# Autodesk Inventor assembly: base mg996r 3mm with top
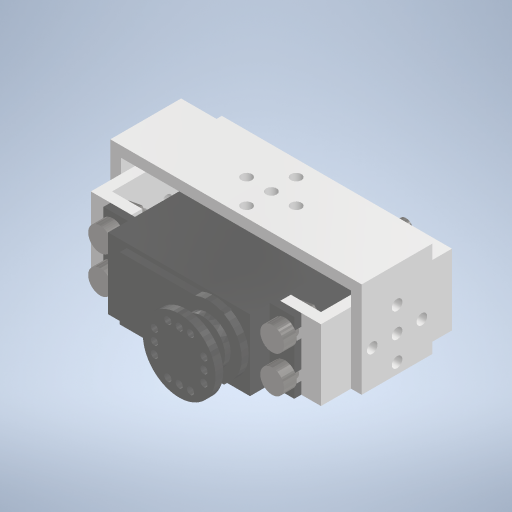
[picture p0: Inventor's stored thumbnail of the model, 512x512]
Saved by Autodesk Inventor 2023 (Build 270158000, 158)
## iProperties
Created: 2022-06-29
Part Number: base mg996r 3mm with top
Document SubType Name: Assembly
Designer: isamu
Author: isamu
## iProperties of the stored document servo frame part 004.ipt
Created: 2022-06-29
Part Number: servo frame part 004
Material: Generic
Document SubType Name: Modeling
Designer: isamu
Density: 1 g/cm^3
Appearance: Default
Author: isamu
## iProperties of the stored document servo frame part 3.iam
Created: 2022-06-29
Part Number: servo frame part 3
Description: FreeCAD Model
Document SubType Name: Assembly
Designer: isamu
Authority: Unknown
Title: Open CASCADE Shape Model
Author: Author
Sending System: FreeCAD
Preprocessor: Open CASCADE STEP processor 7.5
## Documents named in this file (5)
- **D:\personal_projects\robot\inventor\base mg996r 3mm with top.iam*LocalDocs*xAaaaa3caAaaaaaaaAaaaqro0He*servo frame part 004.ipt
- **D:\personal_projects\robot\inventor\base mg996r 3mm with top.iam*LocalDocs*xAaaaqqaaAaaaaaaaAaaaqcqkKd*servo frame part 3.iam
- D:\personal_projects\robot\inventor\base mg996r 3mm with top.iam
- D:\personal_projects\robot\inventor\base mg996r 3mm frame.iam
- D:\personal_projects\robot\exports\frames\servo frame part 3.step
## Components (2 placed, 2 different names)
1. servo frame part 3:1 [sub-assembly] — Mate:1, Mate:2, Mate:3
2. base mg996r 3mm frame:1 [sub-assembly] — Mate:1, Mate:2, Mate:3
## Relationships (3: Mate 3)
- Mate:1: servo frame part 3:1 ↔ base mg996r 3mm frame:1
- Mate:2: servo frame part 3:1 ↔ base mg996r 3mm frame:1
- Mate:3: servo frame part 3:1 ↔ base mg996r 3mm frame:1
